# Autodesk Inventor assembly: Knobber
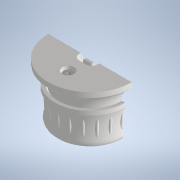
[picture p0: Inventor's stored thumbnail of the model, 180x180]
Saved by Autodesk Inventor 2021 (Build 250183000, 183)
## iProperties
Created: 2024-03-24
Part Number: Knobber
Document SubType Name: Assembly
Designer: Lukas
Author: Lukas
## Documents named in this file (13)
- Z:\Datastorrage\Projects\Knobber\Mechanics\Knobber.iam
- Z:\Datastorrage\Projects\Knobber\Mechanics\XXX.XXXXPCB_Assy_Revision_Knobber.iam
- Z:\Datastorrage\Projects\Knobber\Mechanics\ML2204B 2204-260kv.ipt
- Z:\Datastorrage\Projects\Knobber\Mechanics\Spacerplate.ipt
- Z:\Datastorrage\Projects\Knobber\Mechanics\Baseplate.ipt
- Z:\Datastorrage\Projects\Knobber\Mechanics\M3x12.ipt
- Z:\Datastorrage\Projects\Knobber\Mechanics\M2x4.ipt
- Z:\Datastorrage\Projects\Knobber\Mechanics\Griff.ipt
- Z:\Datastorrage\Projects\Knobber\Mechanics\Magnethalter.ipt
- Z:\Datastorrage\Projects\Knobber\Mechanics\Baseplate_Debug.ipt
- Z:\Datastorrage\Projects\Knobber\Mechanics\PCB_Assy_Revision_Knobber_B.ipt
- Z:\Datastorrage\Projects\Knobber\Mechanics\Button_Extender.ipt
- Z:\Datastorrage\Projects\Knobber\Mechanics\61300411021.ipt
## Components (21 placed, 12 different names)
1. XXX.XXXXPCB_Assy_Revision_Knobber:1 [sub-assembly] — Mate:1, Flush:1, Flush:2, Flush:3, Mate:2, Mate:3, Mate:4, Mate:5, Mate:6, Mate:7
2. PCB_Assy_Revision_Knobber_B:1 — Mate:11, Mate:12, Mate:13, Mate:17, Flush:7, Flush:8
3. ML2204B 2204-260kv:1 — Mate:1, Angle:1, Mate:8, Mate:9, Mate:10, Angle:9, Insert:12, Angle:14
4. Spacerplate:1 — Mate:2, Mate:3, Mate:4, Insert:4, Insert:5, Insert:6, Insert:7, Mate:10, Mate:11
5. Baseplate:1 — Mate:5, Mate:6, Mate:7, Insert:1, Insert:2, Insert:3, Flush:4, Flush:5, Flush:6, Mate:14, Mate:15, Mate:16
6. Baseplate_Debug:1 — Flush:4, Flush:5, Flush:6
7. Griff:1 — Mate:8, Mate:9, Angle:9, Insert:8, Insert:9, Insert:10, Insert:11, Angle:13
8. Magnethalter:1 — Insert:12, Angle:14
9. Button_Extender:1 — Mate:14, Mate:15, Mate:16
10. 61300411021:1 — Mate:17, Flush:7, Flush:8
11. M3x12:1 — Insert:1, Angle:7, Angle:8
12. M3x12:2 — Insert:2, Angle:6, Angle:7, Mate:12
13. M3x12:3 — Insert:3, Angle:5, Angle:6, Mate:13
14. M2x4:1 — Insert:4, Angle:4, Angle:5
15. M2x4:2 — Insert:5, Angle:3, Angle:4
16. M2x4:3 — Insert:6, Angle:2, Angle:3
17. M2x4:4 — Insert:7, Angle:2
18. M2x4:5 — Insert:8, Angle:12, Angle:13
19. M2x4:6 — Insert:9, Angle:11, Angle:12
20. M2x4:7 — Insert:10, Angle:10, Angle:11
21. M2x4:8 — Insert:11, Angle:10
## Relationships (51: Mate 17, Angle 14, Insert 12, Flush 8)
- Mate:1: XXX.XXXXPCB_Assy_Revision_Knobber:1 ↔ ML2204B 2204-260kv:1
- Flush:1: XXX.XXXXPCB_Assy_Revision_Knobber:1
- Flush:2: XXX.XXXXPCB_Assy_Revision_Knobber:1
- Flush:3: XXX.XXXXPCB_Assy_Revision_Knobber:1
- Angle:1 (-90 deg): ML2204B 2204-260kv:1
- Mate:2: XXX.XXXXPCB_Assy_Revision_Knobber:1 ↔ Spacerplate:1
- Mate:3: XXX.XXXXPCB_Assy_Revision_Knobber:1 ↔ Spacerplate:1
- Mate:4: XXX.XXXXPCB_Assy_Revision_Knobber:1 ↔ Spacerplate:1
- Mate:5: XXX.XXXXPCB_Assy_Revision_Knobber:1 ↔ Baseplate:1
- Mate:6: XXX.XXXXPCB_Assy_Revision_Knobber:1 ↔ Baseplate:1
- Mate:7: XXX.XXXXPCB_Assy_Revision_Knobber:1 ↔ Baseplate:1
- Insert:1: Baseplate:1 ↔ M3x12:1
- Insert:2: Baseplate:1 ↔ M3x12:2
- Insert:3: Baseplate:1 ↔ M3x12:3
- Insert:4: Spacerplate:1 ↔ M2x4:1
- Insert:5: Spacerplate:1 ↔ M2x4:2
- Insert:6: Spacerplate:1 ↔ M2x4:3
- Insert:7: Spacerplate:1 ↔ M2x4:4
- Angle:2 (0 deg): M2x4:3 ↔ M2x4:4
- Angle:3 (0 deg): M2x4:2 ↔ M2x4:3
- Angle:4 (0 deg): M2x4:1 ↔ M2x4:2
- Angle:5 (0 deg): M3x12:3 ↔ M2x4:1
- Angle:6 (0 deg): M3x12:2 ↔ M3x12:3
- Angle:7 (0 deg): M3x12:1 ↔ M3x12:2
- Angle:8 (0 deg): M3x12:1
- Mate:8: ML2204B 2204-260kv:1 ↔ Griff:1
- Mate:9: ML2204B 2204-260kv:1 ↔ Griff:1
- Mate:10: ML2204B 2204-260kv:1 ↔ Spacerplate:1
- Angle:9 (0 deg): ML2204B 2204-260kv:1 ↔ Griff:1
- Insert:8: Griff:1 ↔ M2x4:5
- Insert:9: Griff:1 ↔ M2x4:6
- Insert:10: Griff:1 ↔ M2x4:7
- Insert:11: Griff:1 ↔ M2x4:8
- Angle:10 (0 deg): M2x4:7 ↔ M2x4:8
- Angle:11 (0 deg): M2x4:6 ↔ M2x4:7
- Angle:12 (0 deg): M2x4:5 ↔ M2x4:6
- Angle:13 (0 deg): Griff:1 ↔ M2x4:5
- Insert:12: ML2204B 2204-260kv:1 ↔ Magnethalter:1
- Angle:14 (0 deg): ML2204B 2204-260kv:1 ↔ Magnethalter:1
- Flush:4: Baseplate:1 ↔ Baseplate_Debug:1
- Flush:5: Baseplate:1 ↔ Baseplate_Debug:1
- Flush:6: Baseplate:1 ↔ Baseplate_Debug:1
- Mate:11: PCB_Assy_Revision_Knobber_B:1 ↔ Spacerplate:1
- Mate:12: PCB_Assy_Revision_Knobber_B:1 ↔ M3x12:2
- Mate:13: PCB_Assy_Revision_Knobber_B:1 ↔ M3x12:3
- Mate:14 (0.1 mm): Baseplate:1 ↔ Button_Extender:1
- Mate:15 (0.1 mm): Baseplate:1 ↔ Button_Extender:1
- Mate:16 (0.1 mm): Baseplate:1 ↔ Button_Extender:1
- Mate:17: PCB_Assy_Revision_Knobber_B:1 ↔ 61300411021:1
- Flush:7: PCB_Assy_Revision_Knobber_B:1 ↔ 61300411021:1
- Flush:8: PCB_Assy_Revision_Knobber_B:1 ↔ 61300411021:1
